# Autodesk Inventor assembly: Assembly99
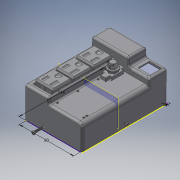
[picture p0: Inventor's stored thumbnail of the model, 180x180]
Saved by Autodesk Inventor 2019 (Build 230136000, 136)
## iProperties
Created: 2019-02-05
Part Number: Assembly99
Document SubType Name: Assembly
Designer: Jorian Bruslind
Author: Jorian Bruslind
## Documents named in this file (8)
- C:\Users\Jorian Bruslind\Documents\GitHub\SchoolWork\ECE341\Final Project\Case\Assembly99.iam
- C:\Users\Jorian Bruslind\Documents\GitHub\SchoolWork\ECE341\Final Project\Case\Case_Top.ipt
- C:\Users\Jorian Bruslind\Documents\GitHub\SchoolWork\ECE341\Final Project\PCB Files\MK1.1\Bluetooth Switch\ExportSTEP\Inventor Version\BTSwitch.iam
- C:\Users\Jorian Bruslind\Documents\GitHub\SchoolWork\ECE341\Final Project\Case\Transformer4Dummy.ipt
- C:\Users\Jorian Bruslind\Documents\GitHub\SchoolWork\ECE341\Final Project\Case\IEC320-C14.iam
- C:\Users\Jorian Bruslind\Documents\GitHub\SchoolWork\ECE341\Final Project\Case\Case_Cover.ipt
- C:\Users\Jorian Bruslind\Documents\GitHub\SchoolWork\ECE341\Final Project\Case\M3 Nut.ipt
- C:\Users\Jorian Bruslind\Documents\GitHub\SchoolWork\ECE341\Final Project\Case\M3x12 Philips Screw.ipt
## Components (21 placed, 7 different names)
1. Case_Top:1 — Mate:2, Mate:3, Flush:1, Mate:7, Mate:8, Mate:9, Mate:10, Flush:2, Mate:11, Mate:19, Mate:22, Mate:23, Tangent:1, Mate:24, Mate:25, Mate:26, Mate:27, Mate:28, Mate:29, Mate:31, Mate:33, Mate:35, Mate:37, Mate:40, Mate:41, Mate:42, Mate:43, Mate:44
2. BTSwitch:1 [sub-assembly] — Mate:2, Mate:3, Mate:10
3. Transformer4Dummy:1 — Mate:7, Mate:8, Mate:9
4. IEC320-C14:1 [sub-assembly] — Flush:1, Mate:13, Flush:3
5. Case_Cover:1 — Flush:2, Mate:11, Mate:13, Flush:3, Mate:30, Mate:34
6. M3 Nut:1 — Mate:19, Mate:38
7. M3 Nut:2 — Mate:39, Mate:40
8. M3 Nut:3 — Mate:36, Mate:37
9. M3 Nut:4 — Mate:30, Mate:31, Mate:32
10. M3 Nut:5 — Mate:26, Mate:27
11. M3 Nut:6 — Mate:28, Mate:29
12. M3 Nut:7 — Mate:22, Mate:23, Tangent:1
13. M3 Nut:8 — Mate:24, Mate:25
14. M3x12 Philips Screw:1 — Mate:33, Mate:38
15. M3x12 Philips Screw:2 — Mate:32
16. M3x12 Philips Screw:3 — Mate:35, Mate:39
17. M3x12 Philips Screw:4 — Mate:34, Mate:36
18. M3x12 Philips Screw:5 — Mate:44
19. M3x12 Philips Screw:6 — Mate:41
20. M3x12 Philips Screw:7 — Mate:43
21. M3x12 Philips Screw:8 — Mate:42
## Relationships (36: Mate 32, Flush 3, Tangent 1)
- Mate:2: Case_Top:1 ↔ BTSwitch:1
- Mate:3: Case_Top:1 ↔ BTSwitch:1
- Flush:1 (-2 mm): Case_Top:1 ↔ IEC320-C14:1
- Mate:7: Case_Top:1 ↔ Transformer4Dummy:1
- Mate:8: Case_Top:1 ↔ Transformer4Dummy:1
- Mate:9: Case_Top:1 ↔ Transformer4Dummy:1
- Mate:10: Case_Top:1 ↔ BTSwitch:1
- Flush:2: Case_Top:1 ↔ Case_Cover:1
- Mate:11 (0.5 mm): Case_Top:1 ↔ Case_Cover:1
- Mate:13: IEC320-C14:1 ↔ Case_Cover:1
- Flush:3: IEC320-C14:1 ↔ Case_Cover:1
- Mate:19: Case_Top:1 ↔ M3 Nut:1
- Mate:22: Case_Top:1 ↔ M3 Nut:7
- Mate:23: Case_Top:1 ↔ M3 Nut:7
- Tangent:1: Case_Top:1 ↔ M3 Nut:7
- Mate:24: Case_Top:1 ↔ M3 Nut:8
- Mate:25: Case_Top:1 ↔ M3 Nut:8
- Mate:26: Case_Top:1 ↔ M3 Nut:5
- Mate:27: Case_Top:1 ↔ M3 Nut:5
- Mate:28: Case_Top:1 ↔ M3 Nut:6
- Mate:29: Case_Top:1 ↔ M3 Nut:6
- Mate:30: Case_Cover:1 ↔ M3 Nut:4
- Mate:31: Case_Top:1 ↔ M3 Nut:4
- Mate:32: M3 Nut:4 ↔ M3x12 Philips Screw:2
- Mate:33: Case_Top:1 ↔ M3x12 Philips Screw:1
- Mate:34: Case_Cover:1 ↔ M3x12 Philips Screw:4
- Mate:35: Case_Top:1 ↔ M3x12 Philips Screw:3
- Mate:36: M3 Nut:3 ↔ M3x12 Philips Screw:4
- Mate:37: Case_Top:1 ↔ M3 Nut:3
- Mate:38: M3 Nut:1 ↔ M3x12 Philips Screw:1
- Mate:39: M3 Nut:2 ↔ M3x12 Philips Screw:3
- Mate:40: Case_Top:1 ↔ M3 Nut:2
- Mate:41: Case_Top:1 ↔ M3x12 Philips Screw:6
- Mate:42: Case_Top:1 ↔ M3x12 Philips Screw:8
- Mate:43: Case_Top:1 ↔ M3x12 Philips Screw:7
- Mate:44: Case_Top:1 ↔ M3x12 Philips Screw:5
